# Autodesk Inventor assembly: PID_SIM
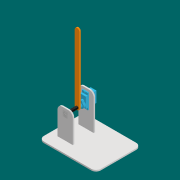
[picture p0: Inventor's stored thumbnail of the model, 180x180]
Saved by Autodesk Inventor 2020.1 (Build 241239000, 239)
## iProperties
Created: 2020-01-27
Part Number: PID_SIM
Document SubType Name: Assembly
Designer: Pluscrafter
Author: Pluscrafter
## Documents named in this file (7)
- C:\Users\Pluscrafter\Documents\serv\PID_SIM.iam
- C:\Users\Pluscrafter\Documents\serv\Servo.ipt
- C:\Users\Pluscrafter\Documents\serv\stab.ipt
- C:\Users\Pluscrafter\Documents\serv\Poti.ipt
- C:\Users\Pluscrafter\Documents\serv\Boden.ipt
- C:\Users\Pluscrafter\Documents\serv\Stutze_Servo.ipt
- C:\Users\Pluscrafter\Documents\serv\Stuze_Poti.ipt
## Components (6 placed, 6 different names)
1. Servo:1 — Mate:1, Mate:5, Mate:6
2. stab:1 — Mate:1, Mate:2, Mate:3, Mate:4
3. Poti:1 — Mate:2, Mate:3, Mate:4, Mate:7, Mate:8, Flush:1
4. Boden:1 — Flush:2, Mate:9, Mate:10
5. Stutze_Servo:1 — Mate:5, Mate:6, Flush:2, Mate:9, Mate:10
6. Stuze_Poti:1 — Mate:7, Mate:8, Flush:1
## Relationships (12: Mate 10, Flush 2)
- Mate:1: Servo:1 ↔ stab:1
- Mate:2: stab:1 ↔ Poti:1
- Mate:3: stab:1 ↔ Poti:1
- Mate:4: stab:1 ↔ Poti:1
- Mate:5: Servo:1 ↔ Stutze_Servo:1
- Mate:6: Servo:1 ↔ Stutze_Servo:1
- Mate:7: Poti:1 ↔ Stuze_Poti:1
- Mate:8: Poti:1 ↔ Stuze_Poti:1
- Flush:1: Poti:1 ↔ Stuze_Poti:1
- Flush:2: Boden:1 ↔ Stutze_Servo:1
- Mate:9: Boden:1 ↔ Stutze_Servo:1
- Mate:10: Boden:1 ↔ Stutze_Servo:1
